# Autodesk Inventor assembly: Assembly
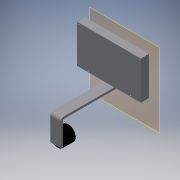
[picture p0: Inventor's stored thumbnail of the model, 180x180]
Saved by Autodesk Inventor 2016 (Build 200138000, 138)
## iProperties
Created: 2016-04-04
Part Number: Assembly
Document SubType Name: Assembly
Designer: Andres
Author: Andres
## Documents named in this file (4)
- \\Mac\Home\Documents\repositorios\MagLev\CAD\Assembly\Assembly.iam
- Z:\Documents\repositorios\MagLev\CAD\Parts\Base.ipt
- Z:\Documents\repositorios\MagLev\CAD\Parts\Brazo.ipt
- Z:\Documents\repositorios\MagLev\CAD\Parts\Coil.ipt
## Components (3 placed, 3 different names)
1. Base:1 — Rigid:1
2. Brazo:1 — Rigid:1, Rigid:2
3. Coil:1 — Rigid:2
## Relationships (2: WeldJoint 2)
- Rigid:1 [WeldJoint]: Base:1 ↔ Brazo:1
- Rigid:2 [WeldJoint]: Brazo:1 ↔ Coil:1
